# Autodesk Inventor assembly: ユニット4
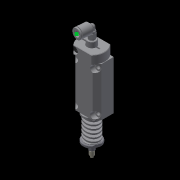
[picture p0: Inventor's stored thumbnail of the model, 180x180]
Saved by Autodesk Inventor 2021.1 (Build 251245000, 245)
## iProperties
Created: 2008-11-13
Document SubType Name: Assembly
Title: ユニット4
## Documents named in this file (9)
- Z:\inventorroom\sample\unit4\unit4 - コピー.iam
- Z:\inventorroom\sample\unit4\WSSM20-10-3.ipt
- Z:\inventorroom\sample\unit4\MHCAW10.ipt
- Z:\inventorroom\sample\unit4\07.ipt
- Z:\inventorroom\sample\unit4\KJL06-M5.ipt
- Z:\inventorroom\sample\unit4\PSPWR10_100_M5_N6_SC10.ipt
- Z:\inventorroom\sample\unit4\SWU17_30.ipt
- Z:\inventorroom\sample\unit4\PSCKNK10-10\PSCKNK10-10.iam
- Z:\inventorroom\sample\unit4\worka.ipt
## Components (8 placed, 8 different names)
1. 07:1 — 挿入:106, 挿入:170
2. KJL06-M5:1 — 挿入:105
3. PSCKNK10-10:1 [sub-assembly] — 挿入:112, 角度:1, メイト:137
4. MHCAW10:1 — 挿入:20, メイト:136, 角度:1, メイト:137
5. WSSM20-10-3:1 — 挿入:20
6. SWU17-30:1 — 挿入:107
7. PSPWR10-100-M5-N6-SC10:1 — 挿入:105, 挿入:106, 挿入:107, メイト:136, 挿入:112
8. worka:1 — 挿入:170
## Relationships (9: Insert 6, Mate 2, Angle 1)
- 挿入:20 [Insert]: MHCAW10:1 ↔ WSSM20-10-3:1
- 挿入:105 [Insert]: KJL06-M5:1 ↔ PSPWR10-100-M5-N6-SC10:1
- 挿入:106 [Insert]: 07:1 ↔ PSPWR10-100-M5-N6-SC10:1
- 挿入:107 [Insert]: SWU17-30:1 ↔ PSPWR10-100-M5-N6-SC10:1
- メイト:136 [Mate]: MHCAW10:1 ↔ PSPWR10-100-M5-N6-SC10:1
- 挿入:112 [Insert] (6 mm): PSCKNK10-10:1 ↔ PSPWR10-100-M5-N6-SC10:1
- 角度:1 [Angle] (0 deg): PSCKNK10-10:1 ↔ MHCAW10:1
- メイト:137 [Mate]: PSCKNK10-10:1 ↔ MHCAW10:1
- 挿入:170 [Insert]: 07:1 ↔ worka:1
